# Autodesk Inventor assembly: Amplifier
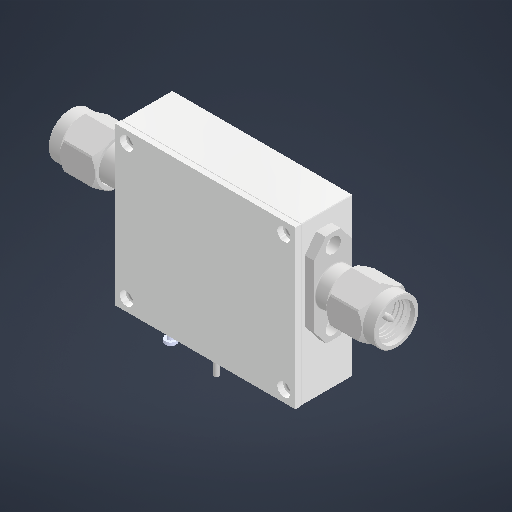
[picture p0: Inventor's stored thumbnail of the model, 512x512]
Saved by Autodesk Inventor 2026.2 (Build 302298010, 298A)
## iProperties
Created: 2026-06-22
Part Number: Amplifier
Document SubType Name: Assembly
Designer: sonata
Author: sonata
## Documents named in this file (6)
- Z:\crush\mechanical\PAM-modules-mount\Amplifier.iam
- Z:\crush\mechanical\PAM-modules-mount\Amplifier Lid ND20.ipt
- Z:\crush\mechanical\PAM-modules-mount\Amplifier Box ND20.ipt
- Z:\crush\mechanical\PAM-modules-mount\PE44032_3D\PE44032_3D\PE44032_3D.ipt
- Z:\crush\mechanical\PAM-modules-mount\1595-2\1595-2\1595-2.ipt
- Z:\crush\mechanical\PAM-modules-mount\FeedThroughCap.ipt
## Components (6 placed, 5 different names)
1. Amplifier Lid ND20:1 — Mate:1, Mate:2, Mate:3
2. Amplifier Box ND20:1 — Mate:1, Mate:2, Mate:3, Mate:4, Mate:5, Mate:6, Mate:7, Mate:8, Mate:9, Mate:10, Mate:11
3. PE44032_3D:1 — Mate:6, Mate:7
4. PE44032_3D:2 — Mate:4, Mate:5
5. 1595-2:1 — Mate:8, Mate:9
6. FeedThroughCap:1 — Mate:10, Mate:11
## Relationships (11: Mate 11)
- Mate:1: Amplifier Lid ND20:1 ↔ Amplifier Box ND20:1
- Mate:2: Amplifier Lid ND20:1 ↔ Amplifier Box ND20:1
- Mate:3: Amplifier Lid ND20:1 ↔ Amplifier Box ND20:1
- Mate:4: Amplifier Box ND20:1 ↔ PE44032_3D:2
- Mate:5: Amplifier Box ND20:1 ↔ PE44032_3D:2
- Mate:6: Amplifier Box ND20:1 ↔ PE44032_3D:1
- Mate:7: Amplifier Box ND20:1 ↔ PE44032_3D:1
- Mate:8: Amplifier Box ND20:1 ↔ 1595-2:1
- Mate:9: Amplifier Box ND20:1 ↔ 1595-2:1
- Mate:10: Amplifier Box ND20:1 ↔ FeedThroughCap:1
- Mate:11: Amplifier Box ND20:1 ↔ FeedThroughCap:1
